# Autodesk Inventor assembly: UpperArm_v2
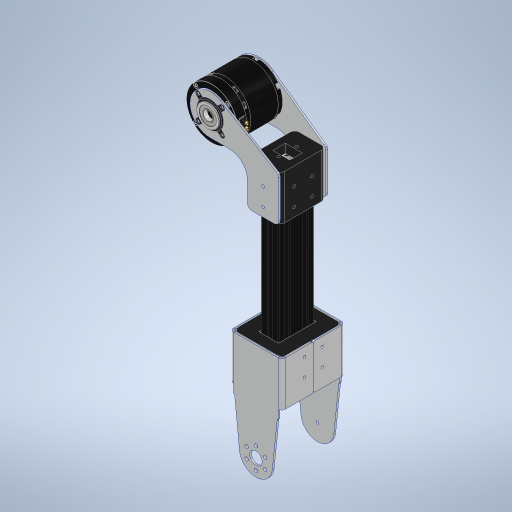
[picture p0: Inventor's stored thumbnail of the model, 512x512]
Saved by Autodesk Inventor 2024.3 (Build 283343010, 343A)
## iProperties
Created: 2025-10-04
Part Number: UpperArm_v2
Document SubType Name: Assembly
Designer: kshau
Author: kshau
## Documents named in this file (13)
- C:\Users\kshau\Documents\inventor\Create_ViperX\Create_ViperX_ALOHA\UpperArm_Component_v2\UpperArm_v2.iam
- C:\Users\kshau\Documents\inventor\Create_ViperX\Create_ViperX_ALOHA\NessesaryParts\HFSB5-2040-200\HFSB5-2040-200\HFSB5-2040-200.ipt
- C:\Users\kshau\Documents\inventor\Create_ViperX\Create_ViperX_ALOHA\UpperArm_Component_v2\framefixpart1_v2.ipt
- C:\Users\kshau\Documents\inventor\Create_ViperX\Create_ViperX_ALOHA\Actuator\RS00\RS00\RS00.iam
- C:\Users\kshau\Documents\inventor\Create_ViperX\Create_ViperX_ALOHA\BasicParts\Bearing\NMB_RF2210X2HH\RF-2210X2HH.iam
- C:\Users\kshau\Documents\inventor\Create_ViperX\Create_ViperX_ALOHA\UpperArm_Component_v2\servoplate1_forR6.ipt
- C:\Users\kshau\Documents\inventor\Create_ViperX\Create_ViperX_ALOHA\UpperArm_Component_v2\servoplate2_forR6.ipt
- C:\Users\kshau\Documents\inventor\Create_ViperX\Create_ViperX_ALOHA\Circuit\XT30(2+2)\XT30(2+2)\XT30(2+2).ipt
- C:\Users\kshau\Documents\inventor\Create_ViperX\Create_ViperX_ALOHA\UpperArm_Component_v2\upperarm_fixplate1_forR0.ipt
- C:\Users\kshau\Documents\inventor\Create_ViperX\Create_ViperX_ALOHA\UpperArm_Component_v2\upperarm_fixplate2_forR0.ipt
- C:\Users\kshau\Documents\inventor\Create_ViperX\Create_ViperX_ALOHA\UpperArm_Component_v2\servohorn_forR0.ipt
- C:\Users\kshau\Documents\inventor\Create_ViperX\Create_ViperX_ALOHA\UpperArm_Component_v2\framefixpart2.ipt
- C:\Users\kshau\Documents\inventor\Create_ViperX\Create_ViperX_ALOHA\UpperArm_Component_v2\servohorn_support_forR0.ipt
## Components (12 placed, 12 different names)
1. framefixpart1_v2:1 — 回転:1, 回転:2, 回転:5, 回転:6, 回転:17, 回転:18
2. framefixpart2:1 — 回転:3, 回転:4, 回転:9, 回転:10, 回転:11, 回転:12
3. HFSB5-2040-200:1 — 回転:1, 回転:2, 回転:3, 回転:4
4. servoplate1_forR6:1 — 回転:5, 回転:6
5. upperarm_fixplate1_forR0:1 — 回転:11, 回転:12, 回転:15, 回転:16
6. upperarm_fixplate2_forR0:1 — 回転:9, 回転:10, 回転:13, 回転:14
7. servohorn_support_forR0:1 — 回転:13, 回転:14, メイト:1, メイト:2
8. RS00:1 [sub-assembly] — 回転:15, 回転:16, メイト:3, メイト:4, メイト:5, メイト:6, メイト:7
9. RF-2210X2HH:1 [sub-assembly] — メイト:1, メイト:2
10. servoplate2_forR6:1 — 回転:17, 回転:18
11. servohorn_forR0:1 — メイト:3, メイト:4
12. XT30(2+2):1 — メイト:5, メイト:6, メイト:7
## Relationships (23: RevoluteJoint 16, Mate 7)
- 回転:1 [RevoluteJoint]: framefixpart1_v2:1 ↔ HFSB5-2040-200:1
- 回転:2 [RevoluteJoint]: framefixpart1_v2:1 ↔ HFSB5-2040-200:1
- 回転:3 [RevoluteJoint]: framefixpart2:1 ↔ HFSB5-2040-200:1
- 回転:4 [RevoluteJoint]: framefixpart2:1 ↔ HFSB5-2040-200:1
- 回転:5 [RevoluteJoint]: framefixpart1_v2:1 ↔ servoplate1_forR6:1
- 回転:6 [RevoluteJoint]: framefixpart1_v2:1 ↔ servoplate1_forR6:1
- 回転:9 [RevoluteJoint]: framefixpart2:1 ↔ upperarm_fixplate2_forR0:1
- 回転:10 [RevoluteJoint]: framefixpart2:1 ↔ upperarm_fixplate2_forR0:1
- 回転:11 [RevoluteJoint]: framefixpart2:1 ↔ upperarm_fixplate1_forR0:1
- 回転:12 [RevoluteJoint]: framefixpart2:1 ↔ upperarm_fixplate1_forR0:1
- 回転:13 [RevoluteJoint]: upperarm_fixplate2_forR0:1 ↔ servohorn_support_forR0:1
- 回転:14 [RevoluteJoint]: upperarm_fixplate2_forR0:1 ↔ servohorn_support_forR0:1
- 回転:15 [RevoluteJoint]: upperarm_fixplate1_forR0:1 ↔ RS00:1
- 回転:16 [RevoluteJoint]: upperarm_fixplate1_forR0:1 ↔ RS00:1
- メイト:1 [Mate]: servohorn_support_forR0:1 ↔ RF-2210X2HH:1
- メイト:2 [Mate]: servohorn_support_forR0:1 ↔ RF-2210X2HH:1
- 回転:17 [RevoluteJoint]: framefixpart1_v2:1 ↔ servoplate2_forR6:1
- 回転:18 [RevoluteJoint]: framefixpart1_v2:1 ↔ servoplate2_forR6:1
- メイト:3 [Mate]: RS00:1 ↔ servohorn_forR0:1
- メイト:4 [Mate]: RS00:1 ↔ servohorn_forR0:1
- メイト:5 [Mate]: RS00:1 ↔ XT30(2+2):1
- メイト:6 [Mate]: RS00:1 ↔ XT30(2+2):1
- メイト:7 [Mate]: RS00:1 ↔ XT30(2+2):1
